# Autodesk Inventor assembly: shaft and nut
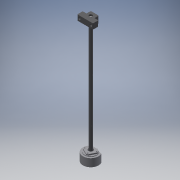
[picture p0: Inventor's stored thumbnail of the model, 180x180]
Saved by Autodesk Inventor 2018 (Build 220112000, 112)
## iProperties
Created: 2017-06-20
Part Number: shaft and nut
Document SubType Name: Assembly
Designer: M228544
Author: M228544
## Documents named in this file (5)
- C:\Users\P301319\Documents\GitHub\CNC-Lathe-CAD\CNC Lathe Project\Project Files\X-axis Changes\X Axis Shaft Assembly\short shaft x axis\shaft and nut.iam
- C:\Users\P301319\Documents\GitHub\CNC-Lathe-CAD\CNC Lathe Project\Project Files\X-axis Changes\X Axis Shaft Assembly\short shaft x axis\shaft.ipt
- C:\Users\P301319\Documents\GitHub\CNC-Lathe-CAD\CNC Lathe Project\Project Files\X-axis Changes\X Axis Shaft Assembly\short shaft x axis\EK 10.ipt
- C:\Users\P301319\Documents\GitHub\CNC-Lathe-CAD\CNC Lathe Project\Project Files\X-axis Changes\X Axis Shaft Assembly\short shaft x axis\FF 10 Part2.ipt
- C:\Users\P301319\Documents\GitHub\CNC-Lathe-CAD\CNC Lathe Project\Project Files\X-axis Changes\X Axis Shaft Assembly\Rosses spaces and ball screw bearing.iam
## Components (4 placed, 4 different names)
1. shaft:1 — Mate:2, Mate:3, Mate:4, Mate:6, Mate:7, Mate:11
2. EK 10:1 — Mate:2, Mate:3, Mate:7, Mate:10, Flush:1, Flush:2
3. FF 10 Part2:1 — Mate:4, Mate:6, Flush:3
4. Rosses spaces and ball screw bearing:1 [sub-assembly] — Angle:1, Mate:11, Flush:3
## Relationships (11: Mate 7, Flush 3, Angle 1)
- Mate:2: shaft:1 ↔ EK 10:1
- Mate:3: shaft:1 ↔ EK 10:1
- Mate:4: shaft:1 ↔ FF 10 Part2:1
- Mate:6: shaft:1 ↔ FF 10 Part2:1
- Mate:7: shaft:1 ↔ EK 10:1
- Mate:10: EK 10:1
- Flush:1: EK 10:1
- Flush:2: EK 10:1
- Angle:1 (0 deg): Rosses spaces and ball screw bearing:1
- Mate:11: shaft:1 ↔ Rosses spaces and ball screw bearing:1
- Flush:3 (-11.55 mm): FF 10 Part2:1 ↔ Rosses spaces and ball screw bearing:1
